# Autodesk Inventor assembly: castor_1inch
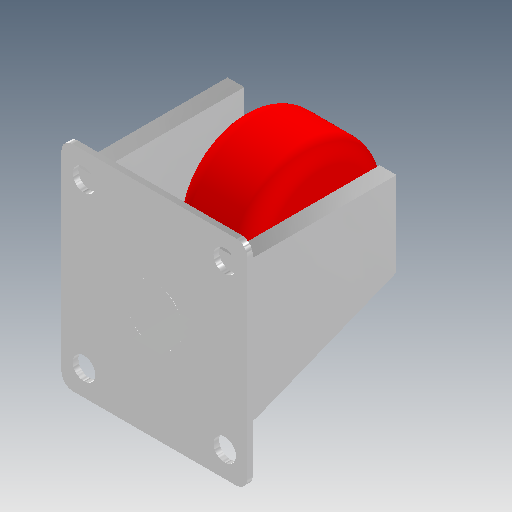
[picture p0: Inventor's stored thumbnail of the model, 512x512]
Saved by Autodesk Inventor 2020 (Build 240168000, 168)
## iProperties
Created: 2020-09-09
Part Number: castor_1inch
Document SubType Name: Assembly
Designer: 이호석
Mass: 24.2859 g
Surface Area: 88.1687 cm^2
Volume: 12.3836 cm^3
Density: 1.96113 g/cm^3
Author: 이호석
## Documents named in this file (4)
- C:\Inventor\Embedded_contest\castor\castor_1inch.iam
- C:\Inventor\Embedded_contest\castor\castor_top.ipt
- C:\Inventor\Embedded_contest\castor\castor_wheel.ipt
- C:\Inventor\Embedded_contest\castor\castor_link2.ipt
## Components (3 placed, 3 different names)
1. castor_top:1 — 삽입:1
2. castor_wheel:1 — 삽입:2, 삽입:3
3. castor_link2:1 — 삽입:1, 삽입:2, 삽입:3
## Relationships (3: Insert 3)
- 삽입:1 [Insert]: castor_top:1 ↔ castor_link2:1
- 삽입:2 [Insert] (5 mm): castor_wheel:1 ↔ castor_link2:1
- 삽입:3 [Insert] (5 mm): castor_wheel:1 ↔ castor_link2:1
